# Autodesk Inventor assembly: Assembly
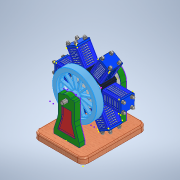
[picture p0: Inventor's stored thumbnail of the model, 180x180]
Saved by Autodesk Inventor 2020 (Build 240168000, 168)
## iProperties
Created: 2021-07-08
Part Number: Assembly
Document SubType Name: Assembly
Designer: lokes
Author: lokes
## Documents named in this file (27)
- C:\Users\lokes\OneDrive\Desktop\major\Assembly.iam
- C:\Users\lokes\OneDrive\Desktop\major\stand.ipt
- C:\Users\lokes\OneDrive\Desktop\major\bearing stand.ipt
- C:\Users\lokes\OneDrive\Desktop\major\bearing holder.ipt
- C:\Users\lokes\OneDrive\Documents\Inventor\Content Center Files\R2020\en-US\BS 4168(1)\BS 4168 - M10 x 25(1).ipt
- C:\Users\lokes\OneDrive\Desktop\major\VALVE HOUSING.ipt
- C:\Users\lokes\OneDrive\Desktop\major\crankcase.ipt
- C:\Users\lokes\OneDrive\Desktop\major\crankcase gasket.ipt
- C:\Users\lokes\OneDrive\Desktop\major\crankcase cover.ipt
- C:\Users\lokes\OneDrive\Desktop\major\CYLINDER.ipt
- C:\Users\lokes\OneDrive\Desktop\major\cylinder head gasket.ipt
- C:\Users\lokes\OneDrive\Desktop\major\cylinder head.ipt
- C:\Users\lokes\OneDrive\Desktop\major\CYLINDER HEAD BOLT.ipt
- C:\Users\lokes\OneDrive\Documents\Inventor\Content Center Files\R2020\en-US\DIN 1587\DIN 1587 - M6 x 1.ipt
- C:\Users\lokes\OneDrive\Documents\Inventor\Content Center Files\R2020\en-US\BS 4168(1)\BS 4168 - M6 x 45(1).ipt
- C:\Users\lokes\OneDrive\Desktop\major\assembly crankshaft.iam
- C:\Users\lokes\OneDrive\Desktop\major\flywheel.ipt
- C:\Users\lokes\OneDrive\Desktop\major\connecting rod hub.ipt
- C:\Users\lokes\OneDrive\Desktop\major\VALVE.ipt
- C:\Users\lokes\OneDrive\Desktop\major\connecting rod.ipt
- C:\Users\lokes\OneDrive\Desktop\major\ASSEMBLY PISTON.iam
- C:\Users\lokes\OneDrive\Documents\Inventor\Content Center Files\R2020\en-US\DIN 472(1)\DIN 472 - 28 x 1.2.ipt
- C:\Users\lokes\OneDrive\Documents\Inventor\Content Center Files\R2020\en-US\DIN BEARING(1)\DIN 625 SKF - SKF 6001.ipt
- C:\Users\lokes\OneDrive\Documents\Inventor\Content Center Files\R2020\en-US\ISO 2338(2)\ISO 2338 - 5 h8 x 16.ipt
- C:\Users\lokes\OneDrive\Documents\Inventor\Content Center Files\R2020\en-US\ISO 7045  H\ISO 7045 - M6 x 16 - 4.8 - H - ISO.ipt
- C:\Users\lokes\OneDrive\Documents\Inventor\Content Center Files\R2020\en-US\Parker HB 125HBL\Parker Hose Barb to Male Pipe 125HBL 125HBL-4-2.ipt
- C:\Users\lokes\OneDrive\Documents\Inventor\Content Center Files\R2020\en-US\SS-ISO 4028\ISO 4028 - M5 x 8SS-ISO.ipt
## Components (120 placed, 26 different names)
1. stand:1 — Mate:1, Mate:2, Mate:6, Mate:7, Mate:8, Mate:9, Mate:16, Mate:57, Mate:58, Mate:59, Mate:60, Mate:61, Mate:62, Mate:64
2. bearing stand:1 — Mate:1, Mate:2, Mate:16, Mate:18, Mate:19, Mate:21, Mate:44, Mate:45, Mate:110
3. BS 4168 : Part 1 Hexagon Socket Head Cap Screw - Metric M10 x 25:1 — Mate:6, Mate:7
4. BS 4168 : Part 1 Hexagon Socket Head Cap Screw - Metric M10 x 25:2 — Mate:8, Mate:9
5. VALVE HOUSING:1 — Mate:18, Mate:19, Mate:20, Mate:22, Mate:69, Mate:111
6. crankcase gasket:1 — Mate:23, Mate:24, Mate:26
7. crankcase cover:1 — Mate:26, Mate:27, Mate:65, Mate:109
8. assembly crankshaft:1 [sub-assembly] — Mate:51, Mate:52, Rotation:1, Mate:55, Mate:56, Mate:63, Mate:68, Mate:69, Mate:93, Mate:94, Tangent:1
9. flywheel:1 — Rotation:1, Mate:55, Mate:63, Mate:65, Mate:112
10. connecting rod hub:1 — Mate:51, Mate:66, Mate:67, Mate:68, Mate:72, Mate:73, Mate:76, Mate:77, Mate:80, Mate:81, Mate:84, Mate:85, Mate:88, Mate:89, Mate:97, Mate:99, Mate:100, Mate:101, Mate:102, Mate:103, Mate:104, Mate:105, Mate:106, Mate:107
11. VALVE:1 — Mate:52, Mate:53
12. bearing holder:1 — Mate:56, Mate:57, Mate:58, Mate:64, Mate:92, Mate:95
13. BS 4168 : Part 1 Hexagon Socket Head Cap Screw - Metric M10 x 25:3 — Mate:59, Mate:60
14. BS 4168 : Part 1 Hexagon Socket Head Cap Screw - Metric M10 x 25:4 — Mate:61, Mate:62
15. connecting rod:1 — Mate:66, Mate:67, Mate:70
16. ASSEMBLY PISTON:1 [sub-assembly] — Mate:90, Mate:91
17. ASSEMBLY PISTON:2 [sub-assembly] — Mate:86, Mate:87
18. ASSEMBLY PISTON:3 [sub-assembly] — Mate:82, Mate:83
19. ASSEMBLY PISTON:4 [sub-assembly] — Mate:74, Mate:75
20. ASSEMBLY PISTON:5 [sub-assembly] — Mate:70, Mate:71
21. ASSEMBLY PISTON:6 [sub-assembly] — Mate:78, Mate:79
22. connecting rod:2 — Mate:76, Mate:77, Mate:78, Mate:98
23. connecting rod:3 — Mate:72, Mate:73, Mate:74
24. connecting rod:5 — Mate:84, Mate:85, Mate:86
25. connecting rod:6 — Mate:80, Mate:81, Mate:82, Mate:96
26. connecting rod:8 — Mate:88, Mate:89, Mate:90
27. DIN 472 28 x 1.2:1 — Mate:92, Mate:93
28. DIN 625 SKF SKF 6001:1 — Mate:94, Mate:95
29. ISO 2338 5 h8 x 16:1 — Mate:98, Mate:99
30. ISO 2338 5 h8 x 16:2 — Mate:96, Mate:97
31. ISO 2338 5 h8 x 16:3 — Mate:100, Mate:101
32. ISO 2338 5 h8 x 16:4 — Mate:102, Mate:103
33. ISO 2338 5 h8 x 16:5 — Mate:104, Mate:105
34. ISO 2338 5 h8 x 16:6 — Mate:106, Mate:107
35. Parker Hose Barb to Male Pipe 125HBL 125HBL-4-2:1 — Mate:110, Mate:111
36. SS ISO 4028 M5 x 8:1 — Mate:112, Tangent:1
37. cylinder head:1 — Mate:37, Mate:38, Mate:39, Mate:42, Mate:43
38. cylinder head gasket:1 — Mate:32, Mate:33, Mate:35, Mate:36, Mate:37, Mate:71
39. CYLINDER:1 — Mate:29, Mate:30, Mate:31, Mate:32, Mate:33, Mate:35, Mate:36, Mate:38, Mate:39
40. cylinder head:2
41. cylinder head gasket:2 — Mate:79
42. CYLINDER:2
43. cylinder head:3
44. cylinder head gasket:3 — Mate:83
45. CYLINDER:3
46. cylinder head:4
47. cylinder head gasket:4 — Mate:87
48. CYLINDER:4
49. cylinder head:5
50. cylinder head gasket:5 — Mate:91
51. CYLINDER:5
52. cylinder head:6
53. cylinder head gasket:6 — Mate:75
54. CYLINDER:6
55. BS 4168 : Part 1 Hexagon Socket Head Cap Screw - Metric M6 x 45:2 — Mate:44, Mate:45
56. BS 4168 : Part 1 Hexagon Socket Head Cap Screw - Metric M6 x 45:7
57. BS 4168 : Part 1 Hexagon Socket Head Cap Screw - Metric M6 x 45:8
58. BS 4168 : Part 1 Hexagon Socket Head Cap Screw - Metric M6 x 45:9
59. BS 4168 : Part 1 Hexagon Socket Head Cap Screw - Metric M6 x 45:10
60. BS 4168 : Part 1 Hexagon Socket Head Cap Screw - Metric M6 x 45:11
61. ISO 7045 H M6 x 16 - 4.8 - H:1 — Mate:108, Mate:109
62. crankcase:1 — Mate:20, Mate:21, Mate:22, Mate:23, Mate:24, Mate:27, Mate:29, Mate:30, Mate:31, Mate:53, Mate:108
63. ISO 7045 H M6 x 16 - 4.8 - H:7
64. crankcase:2
65. ISO 7045 H M6 x 16 - 4.8 - H:8
66. crankcase:3
67. ISO 7045 H M6 x 16 - 4.8 - H:9
68. crankcase:4
69. ISO 7045 H M6 x 16 - 4.8 - H:10
70. crankcase:5
71. ISO 7045 H M6 x 16 - 4.8 - H:11
72. crankcase:6
73. DIN 1587 M6:1 — Mate:40, Mate:41, Mate:42
74. CYLINDER HEAD BOLT:4 — Mate:40, Mate:41, Mate:43
75. DIN 1587 M6:2
76. CYLINDER HEAD BOLT:5
77. DIN 1587 M6:3
78. CYLINDER HEAD BOLT:6
79. DIN 1587 M6:4
80. CYLINDER HEAD BOLT:7
81. DIN 1587 M6:5
82. CYLINDER HEAD BOLT:8
83. DIN 1587 M6:6
84. CYLINDER HEAD BOLT:9
85. DIN 1587 M6:7
86. CYLINDER HEAD BOLT:10
87. DIN 1587 M6:8
88. CYLINDER HEAD BOLT:11
89. DIN 1587 M6:9
90. CYLINDER HEAD BOLT:12
91. DIN 1587 M6:10
92. CYLINDER HEAD BOLT:13
93. DIN 1587 M6:11
94. CYLINDER HEAD BOLT:14
95. DIN 1587 M6:12
96. CYLINDER HEAD BOLT:15
97. DIN 1587 M6:13
98. CYLINDER HEAD BOLT:16
99. DIN 1587 M6:14
100. CYLINDER HEAD BOLT:17
101. DIN 1587 M6:15
102. CYLINDER HEAD BOLT:18
103. DIN 1587 M6:16
104. CYLINDER HEAD BOLT:19
105. DIN 1587 M6:17
106. CYLINDER HEAD BOLT:20
107. DIN 1587 M6:18
108. CYLINDER HEAD BOLT:21
109. DIN 1587 M6:19
110. CYLINDER HEAD BOLT:22
111. DIN 1587 M6:20
112. CYLINDER HEAD BOLT:23
113. DIN 1587 M6:21
114. CYLINDER HEAD BOLT:24
115. DIN 1587 M6:22
116. CYLINDER HEAD BOLT:25
117. DIN 1587 M6:23
118. CYLINDER HEAD BOLT:26
119. DIN 1587 M6:24
120. CYLINDER HEAD BOLT:27
## Component patterns: (6 elements, first: cylinder head:1 + cylinder head gasket:1 + CYLINDER:1), (6 elements, first: BS 4168 : Part 1 Hexagon Socket Head Cap Screw - Metric M6 x 45:2), (6 elements, first: ISO 7045 H M6 x 16 - 4.8 - H:1 + crankcase:1), (4 elements, first: DIN 1587 M6:1 + CYLINDER HEAD BOLT:4), Component Pattern 1:2 (4 elements), Component Pattern 1:3 (4 elements), Component Pattern 1:4 (4 elements), Component Pattern 1:5 (4 elements), Component Pattern 1:6 (4 elements)
## Relationships (95: Mate 93, RelateRotation 1, Tangent 1)
- Mate:1: stand:1 ↔ bearing stand:1
- Mate:2: stand:1 ↔ bearing stand:1
- Mate:6: stand:1 ↔ BS 4168 : Part 1 Hexagon Socket Head Cap Screw - Metric M10 x 25:1
- Mate:7: stand:1 ↔ BS 4168 : Part 1 Hexagon Socket Head Cap Screw - Metric M10 x 25:1
- Mate:8: stand:1 ↔ BS 4168 : Part 1 Hexagon Socket Head Cap Screw - Metric M10 x 25:2
- Mate:9: stand:1 ↔ BS 4168 : Part 1 Hexagon Socket Head Cap Screw - Metric M10 x 25:2
- Mate:16: stand:1 ↔ bearing stand:1
- Mate:18: bearing stand:1 ↔ VALVE HOUSING:1
- Mate:19: bearing stand:1 ↔ VALVE HOUSING:1
- Mate:20: VALVE HOUSING:1 ↔ crankcase:1
- Mate:21: bearing stand:1 ↔ crankcase:1
- Mate:22: VALVE HOUSING:1 ↔ crankcase:1
- Mate:23: crankcase gasket:1 ↔ crankcase:1
- Mate:24: crankcase gasket:1 ↔ crankcase:1
- Mate:26: crankcase gasket:1 ↔ crankcase cover:1
- Mate:27: crankcase cover:1 ↔ crankcase:1
- Mate:29: CYLINDER:1 ↔ crankcase:1
- Mate:30: CYLINDER:1 ↔ crankcase:1
- Mate:31: CYLINDER:1 ↔ crankcase:1
- Mate:32: cylinder head gasket:1 ↔ CYLINDER:1
- Mate:33: cylinder head gasket:1 ↔ CYLINDER:1
- Mate:35: cylinder head gasket:1 ↔ CYLINDER:1
- Mate:36: cylinder head gasket:1 ↔ CYLINDER:1
- Mate:37: cylinder head:1 ↔ cylinder head gasket:1
- Mate:38: cylinder head:1 ↔ CYLINDER:1
- Mate:39: cylinder head:1 ↔ CYLINDER:1
- Mate:40: DIN 1587 M6:1 ↔ CYLINDER HEAD BOLT:4
- Mate:41: DIN 1587 M6:1 ↔ CYLINDER HEAD BOLT:4
- Mate:42: cylinder head:1 ↔ DIN 1587 M6:1
- Mate:43: cylinder head:1 ↔ CYLINDER HEAD BOLT:4
- Mate:44: bearing stand:1 ↔ BS 4168 : Part 1 Hexagon Socket Head Cap Screw - Metric M6 x 45:2
- Mate:45: bearing stand:1 ↔ BS 4168 : Part 1 Hexagon Socket Head Cap Screw - Metric M6 x 45:2
- Mate:51: assembly crankshaft:1 ↔ connecting rod hub:1
- Mate:52: assembly crankshaft:1 ↔ VALVE:1
- Mate:53: VALVE:1 ↔ crankcase:1
- Rotation:1 [RelateRotation] (1 ul): assembly crankshaft:1 ↔ flywheel:1
- Mate:55: assembly crankshaft:1 ↔ flywheel:1
- Mate:56: assembly crankshaft:1 ↔ bearing holder:1
- Mate:57: stand:1 ↔ bearing holder:1
- Mate:58: stand:1 ↔ bearing holder:1
- Mate:59: stand:1 ↔ BS 4168 : Part 1 Hexagon Socket Head Cap Screw - Metric M10 x 25:3
- Mate:60: stand:1 ↔ BS 4168 : Part 1 Hexagon Socket Head Cap Screw - Metric M10 x 25:3
- Mate:61: stand:1 ↔ BS 4168 : Part 1 Hexagon Socket Head Cap Screw - Metric M10 x 25:4
- Mate:62: stand:1 ↔ BS 4168 : Part 1 Hexagon Socket Head Cap Screw - Metric M10 x 25:4
- Mate:63: assembly crankshaft:1 ↔ flywheel:1
- Mate:64: stand:1 ↔ bearing holder:1
- Mate:65 (2.54 mm): crankcase cover:1 ↔ flywheel:1
- Mate:66: connecting rod hub:1 ↔ connecting rod:1
- Mate:67: connecting rod hub:1 ↔ connecting rod:1
- Mate:68: assembly crankshaft:1 ↔ connecting rod hub:1
- Mate:69: VALVE HOUSING:1 ↔ assembly crankshaft:1
- Mate:70: connecting rod:1 ↔ ASSEMBLY PISTON:5
- Mate:71: ASSEMBLY PISTON:5 ↔ cylinder head gasket:1
- Mate:72: connecting rod hub:1 ↔ connecting rod:3
- Mate:73: connecting rod hub:1 ↔ connecting rod:3
- Mate:74: ASSEMBLY PISTON:4 ↔ connecting rod:3
- Mate:75: ASSEMBLY PISTON:4 ↔ cylinder head gasket:6
- Mate:76: connecting rod hub:1 ↔ connecting rod:2
- Mate:77: connecting rod hub:1 ↔ connecting rod:2
- Mate:78: ASSEMBLY PISTON:6 ↔ connecting rod:2
- Mate:79: ASSEMBLY PISTON:6 ↔ cylinder head gasket:2
- Mate:80: connecting rod hub:1 ↔ connecting rod:6
- Mate:81: connecting rod hub:1 ↔ connecting rod:6
- Mate:82: ASSEMBLY PISTON:3 ↔ connecting rod:6
- Mate:83: ASSEMBLY PISTON:3 ↔ cylinder head gasket:3
- Mate:84: connecting rod hub:1 ↔ connecting rod:5
- Mate:85: connecting rod hub:1 ↔ connecting rod:5
- Mate:86: ASSEMBLY PISTON:2 ↔ connecting rod:5
- Mate:87: ASSEMBLY PISTON:2 ↔ cylinder head gasket:4
- Mate:88: connecting rod hub:1 ↔ connecting rod:8
- Mate:89: connecting rod hub:1 ↔ connecting rod:8
- Mate:90: ASSEMBLY PISTON:1 ↔ connecting rod:8
- Mate:91: ASSEMBLY PISTON:1 ↔ cylinder head gasket:5
- Mate:92: bearing holder:1 ↔ DIN 472 28 x 1.2:1
- Mate:93: assembly crankshaft:1 ↔ DIN 472 28 x 1.2:1
- Mate:94: assembly crankshaft:1 ↔ DIN 625 SKF SKF 6001:1
- Mate:95: bearing holder:1 ↔ DIN 625 SKF SKF 6001:1
- Mate:96: connecting rod:6 ↔ ISO 2338 5 h8 x 16:2
- Mate:97: connecting rod hub:1 ↔ ISO 2338 5 h8 x 16:2
- Mate:98: connecting rod:2 ↔ ISO 2338 5 h8 x 16:1
- Mate:99: connecting rod hub:1 ↔ ISO 2338 5 h8 x 16:1
- Mate:100: connecting rod hub:1 ↔ ISO 2338 5 h8 x 16:3
- Mate:101: connecting rod hub:1 ↔ ISO 2338 5 h8 x 16:3
- Mate:102: connecting rod hub:1 ↔ ISO 2338 5 h8 x 16:4
- Mate:103: connecting rod hub:1 ↔ ISO 2338 5 h8 x 16:4
- Mate:104: connecting rod hub:1 ↔ ISO 2338 5 h8 x 16:5
- Mate:105: connecting rod hub:1 ↔ ISO 2338 5 h8 x 16:5
- Mate:106: connecting rod hub:1 ↔ ISO 2338 5 h8 x 16:6
- Mate:107: connecting rod hub:1 ↔ ISO 2338 5 h8 x 16:6
- Mate:108: ISO 7045 H M6 x 16 - 4.8 - H:1 ↔ crankcase:1
- Mate:109: crankcase cover:1 ↔ ISO 7045 H M6 x 16 - 4.8 - H:1
- Mate:110: bearing stand:1 ↔ Parker Hose Barb to Male Pipe 125HBL 125HBL-4-2:1
- Mate:111: VALVE HOUSING:1 ↔ Parker Hose Barb to Male Pipe 125HBL 125HBL-4-2:1
- Mate:112: flywheel:1 ↔ SS ISO 4028 M5 x 8:1
- Tangent:1: assembly crankshaft:1 ↔ SS ISO 4028 M5 x 8:1
